# Autodesk Inventor assembly: Gelenk
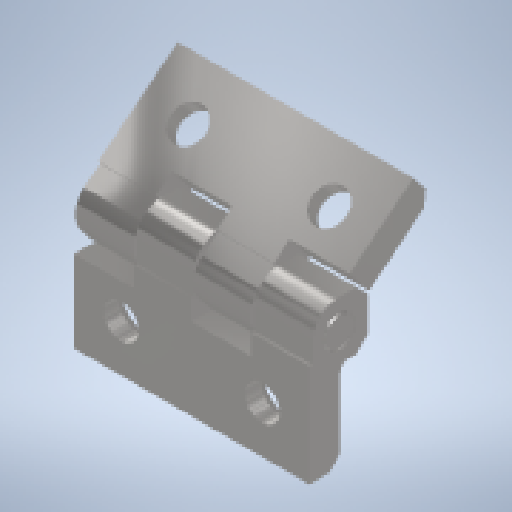
[picture p0: Inventor's stored thumbnail of the model, 512x512]
Saved by Autodesk Inventor 2024.4 (Build 284460000, 460)
## iProperties
Created: 2026-01-17
Part Number: Gelenk
Description: Gelenk
Document SubType Name: Assembly
Designer: Philf
Mass: 103.184 g
Surface Area: 63.606 cm^2
Volume: 12.898 cm^3
Density: 8 g/cm^3
Masse[kg]: 0,103 kg
## Documents named in this file (4)
- C:\Users\Philf\Documents\Vault\Daten\I60-Konstruktion\I60-Gruppe-7\Sitz\Gelenk.iam
- C:\Users\Philf\Documents\Vault\Daten\I60-Konstruktion\I60-Gruppe-7\Sitz\GelenkOT.ipt
- C:\Users\Philf\Documents\Vault\Daten\I60-Konstruktion\I60-Gruppe-7\Sitz\GelenkUT.ipt
- C:\Users\Philf\Documents\Vault\Daten\I60-Konstruktion\I60-Gruppe-7\Sitz\GelenkStift.ipt
## Components (3 placed, 3 different names)
1. GelenkOT:1 — Drehbar:1, Passend:1, Fluchtend:1
2. GelenkUT:1 — Drehbar:1
3. GelenkStift:1 — Passend:1, Fluchtend:1
## Relationships (3: RevoluteJoint 1, Mate 1, Flush 1)
- Drehbar:1 [RevoluteJoint] (-15 mm): GelenkOT:1 ↔ GelenkUT:1
- Passend:1 [Mate]: GelenkOT:1 ↔ GelenkStift:1
- Fluchtend:1 [Flush]: GelenkOT:1 ↔ GelenkStift:1
